# Autodesk Inventor assembly: Ari Tsugi
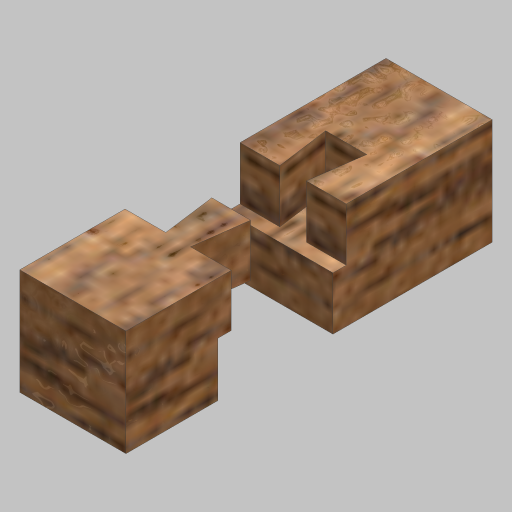
[picture p0: Inventor's stored thumbnail of the model, 512x512]
Saved by Autodesk Inventor 2023 (Build 270158000, 158)
## iProperties
Created: 2026-07-03
Part Number: Ari Tsugi
Document SubType Name: Assembly
Designer: MARTIN MAESTRE
Author: MARTIN MAESTRE
## Documents named in this file (3)
- C:\Users\MARTIN MAESTRE\OneDrive - Universidad de los Andes\POSTGRADO\202610\MAESTRIA\PROBLEMA ESPECIAL\CADS_TOLERANCIAS\Repositorio\Ari Tsugi\Ari Tsugi.iam
- C:\Users\MARTIN MAESTRE\OneDrive - Universidad de los Andes\POSTGRADO\202610\MAESTRIA\PROBLEMA ESPECIAL\CADS_TOLERANCIAS\Repositorio\Ari Tsugi\Part_Female.ipt
- C:\Users\MARTIN MAESTRE\OneDrive - Universidad de los Andes\POSTGRADO\202610\MAESTRIA\PROBLEMA ESPECIAL\CADS_TOLERANCIAS\Repositorio\Ari Tsugi\Part_Male.ipt
## Components (2 placed, 2 different names)
1. Part_Female:1 — Coincidencia:1, Coincidencia:2, Coincidencia:3, Nivelación:1, Nivelación:2
2. Part_Male:1 — Nivelación:1, Nivelación:2
## Relationships (5: Mate 3, Flush 2)
- Coincidencia:1 [Mate]: Part_Female:1
- Coincidencia:2 [Mate]: Part_Female:1
- Coincidencia:3 [Mate]: Part_Female:1
- Nivelación:1 [Flush]: Part_Female:1 ↔ Part_Male:1
- Nivelación:2 [Flush]: Part_Female:1 ↔ Part_Male:1
